# Autodesk Inventor assembly: JewlArm
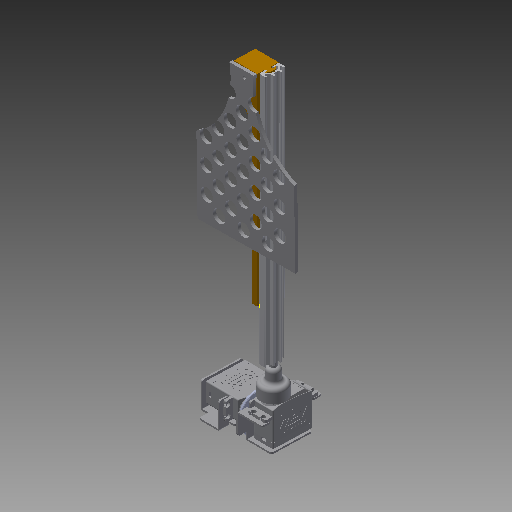
[picture p0: Inventor's stored thumbnail of the model, 512x512]
Saved by Autodesk Inventor 2017 (Build 210142000, 142)
## iProperties
Created: 2017-10-12
Part Number: JewlArm
Document SubType Name: Assembly
Designer: User
Author: User
## Documents named in this file (9)
- C:\Robotics\CAD\2017-18_CAD\Miscellaneous\JewlArm.iam
- C:\Robotics\CAD\COTSParts\Tetrix\Tetrix bracket - single servo.ipt
- C:\Robotics\CAD\2017-18_CAD\FlapperSlapperPlate.ipt
- C:\Robotics\CAD\2017-18_CAD\FlapperSlapper.ipt
- C:\Robotics\CAD\COTSParts\Bosch Extrusion\Bosch 20x20 10in half.ipt
- C:\Robotics\CAD\2017-18_CAD\20X20Connector.ipt
- C:\Robotics\CAD\COTSParts\Rev\REV-41-1097SmartServo.iam
- C:\Robotics\CAD\COTSParts\Rev\REV-41-1363ServoHorn.ipt
- C:\Robotics\CAD\COTSParts\Rev\REV-41-1097SmartServo.ipt
## Components (11 placed, 7 different names)
1. Tetrix bracket - single servo:1 — Insert:1, Insert:2, Angle:1, Insert:9, Angle:3
2. Tetrix bracket - single servo:2 — Insert:3, Insert:4, Insert:5, Insert:7, Angle:1, Angle:2, Insert:11, Angle:4
3. FlapperSlapperPlate:1 — Mate:27, Mate:28, Mate:29
4. FlapperSlapper:1 — Mate:24, Tangent:1, Tangent:2, Insert:8, Insert:12
5. Bosch 20x20 10in half:1 — Mate:24, Tangent:1, Tangent:2, Flush:3, Mate:25, Mate:26, Angle:2
6. 20X20Connector:1 — Flush:3, Mate:25, Mate:26, Mate:27, Mate:28, Mate:29
7. REV-41-1097SmartServo:1 [sub-assembly] — Insert:1, Insert:2, Insert:6
8. REV-41-1097SmartServo:2 [sub-assembly] — Insert:3, Insert:7, Insert:8
9. REV-41-1363ServoHorn:1 — Insert:4, Insert:5, Insert:6, Insert:10
10. REV-41-1097SmartServo:3 — Insert:11, Angle:4, Insert:12
11. REV-41-1097SmartServo:4 — Insert:9, Angle:3, Insert:10
## Relationships (25: Insert 12, Mate 6, Angle 4, Tangent 2, Flush 1)
- Mate:24 (-31.75 mm): FlapperSlapper:1 ↔ Bosch 20x20 10in half:1
- Tangent:1: FlapperSlapper:1 ↔ Bosch 20x20 10in half:1
- Tangent:2: FlapperSlapper:1 ↔ Bosch 20x20 10in half:1
- Flush:3: Bosch 20x20 10in half:1 ↔ 20X20Connector:1
- Mate:25: Bosch 20x20 10in half:1 ↔ 20X20Connector:1
- Mate:26: Bosch 20x20 10in half:1 ↔ 20X20Connector:1
- Mate:27: FlapperSlapperPlate:1 ↔ 20X20Connector:1
- Insert:1 (2.794 mm): Tetrix bracket - single servo:1 ↔ REV-41-1097SmartServo:1
- Insert:2 (2.794 mm): Tetrix bracket - single servo:1 ↔ REV-41-1097SmartServo:1
- Insert:3 (2.794 mm): Tetrix bracket - single servo:2 ↔ REV-41-1097SmartServo:2
- Insert:4: Tetrix bracket - single servo:2 ↔ REV-41-1363ServoHorn:1
- Insert:5: Tetrix bracket - single servo:2 ↔ REV-41-1363ServoHorn:1
- Insert:6: REV-41-1097SmartServo:1 ↔ REV-41-1363ServoHorn:1
- Insert:7 (2.794 mm): Tetrix bracket - single servo:2 ↔ REV-41-1097SmartServo:2
- Insert:8: FlapperSlapper:1 ↔ REV-41-1097SmartServo:2
- Mate:28 (-13.97 mm): FlapperSlapperPlate:1 ↔ 20X20Connector:1
- Mate:29 (-6.731 mm): FlapperSlapperPlate:1 ↔ 20X20Connector:1
- Angle:1 (0 deg): Tetrix bracket - single servo:1 ↔ Tetrix bracket - single servo:2
- Angle:2 (0 deg): Tetrix bracket - single servo:2 ↔ Bosch 20x20 10in half:1
- Insert:9 (-2.794 mm): Tetrix bracket - single servo:1 ↔ REV-41-1097SmartServo:4
- Angle:3 (0 deg): Tetrix bracket - single servo:1 ↔ REV-41-1097SmartServo:4
- Insert:10: REV-41-1363ServoHorn:1 ↔ REV-41-1097SmartServo:4
- Insert:11 (-2.794 mm): Tetrix bracket - single servo:2 ↔ REV-41-1097SmartServo:3
- Angle:4 (0 deg): Tetrix bracket - single servo:2 ↔ REV-41-1097SmartServo:3
- Insert:12: FlapperSlapper:1 ↔ REV-41-1097SmartServo:3
